# Autodesk Inventor assembly: FINAL ASSEMBLY CONNECTORS IN
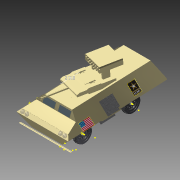
[picture p0: Inventor's stored thumbnail of the model, 180x180]
Saved by Autodesk Inventor 2015 (Build 190159000, 159)
## iProperties
Created: 2015-04-25
Part Number: FINAL ASSEMBLY CONNECTORS IN
Document SubType Name: Assembly
Designer: Simrun
Author: Simrun
## Documents named in this file (11)
- C:\Users\Simrun\Desktop\ALL M1117 Parts\FINAL ASSEMBLY CONNECTORS IN.iam
- C:\Users\Simrun\Desktop\ALL M1117 Parts\Correct middle piece Thursday 16.ipt
- C:\Users\Simrun\Desktop\ALL M1117 Parts\WORKING FRONT PART SPACESHIP COPY.ipt
- C:\Users\Simrun\Desktop\ALL M1117 Parts\T9 One Block Socket.ipt
- C:\Users\Simrun\Desktop\ALL M1117 Parts\T9 Two Block Socket.ipt
- C:\Users\Simrun\Desktop\ALL M1117 Parts\T9 Connector.ipt
- C:\Users\Simrun\Desktop\ALL M1117 Parts\Correct BACK PIECE.ipt
- C:\Users\Simrun\Desktop\ALL M1117 Parts\NewImprovedAxilforWheel.ipt
- C:\Users\Simrun\Desktop\ALL M1117 Parts\New Cannon M117 Guardian (1).ipt
- C:\Users\Simrun\Desktop\ALL M1117 Parts\AFinalWheel.ipt
- C:\Users\Simrun\Desktop\ALL M1117 Parts\Light.ipt
## Components (23 placed, 10 different names)
1. Correct middle piece Thursday 16:1 — Flush:1, Flush:2, Flush:3, Flush:8, Flush:9, Mate:4, Flush:10, Mate:7, Flush:12, Flush:13, Mate:9, Flush:15, Flush:16, Flush:17, Flush:18, Flush:19, Flush:20, Mate:10, Insert:1
2. WORKING FRONT PART SPACESHIP COPY:1 — Mate:1, Flush:4, Flush:5, Mate:3, Flush:8, Flush:9, Mate:4, Flush:10, Insert:3, Insert:6, Insert:11, Insert:12, Insert:13, Insert:14
3. T9 One Block Socket:1 — Flush:1, Flush:2, Flush:3
4. T9 Two Block Socket:1 — Mate:1, Flush:4, Flush:5, Mate:2, Flush:6
5. T9 Connector:1 — Mate:2, Flush:6, Flush:7
6. Correct BACK PIECE:1 — Mate:5, Mate:6, Flush:11, Flush:15, Flush:16, Flush:17, Flush:18, Flush:19, Flush:20, Mate:10, Insert:4, Insert:5
7. T9 Connector:2 — Mate:8, Flush:14, Mate:9
8. T9 One Block Socket:2 — Mate:5, Mate:6, Flush:11
9. T9 Two Block Socket:2 — Mate:7, Flush:12, Flush:13, Mate:8, Flush:14
10. NewImprovedAxilforWheel:1 — Insert:1, Insert:2
11. NewImprovedAxilforWheel:2 — Insert:5, Insert:7
12. NewImprovedAxilforWheel:3 — Insert:6, Insert:8
13. NewImprovedAxilforWheel:4 — Insert:4, Insert:9
14. NewImprovedAxilforWheel:5 — Insert:3, Insert:10
15. New Cannon M117 Guardian (1):1 — Insert:2
16. AFinalWheel:1 — Insert:8
17. AFinalWheel:2 — Insert:7
18. AFinalWheel:3 — Insert:9
19. AFinalWheel:4 — Insert:10
20. Light:1 — Insert:11
21. Light:2 — Insert:12
22. Light:3 — Insert:13
23. Light:4 — Insert:14
## Relationships (44: Flush 20, Insert 14, Mate 10)
- Flush:1: Correct middle piece Thursday 16:1 ↔ T9 One Block Socket:1
- Flush:2: Correct middle piece Thursday 16:1 ↔ T9 One Block Socket:1
- Flush:3: Correct middle piece Thursday 16:1 ↔ T9 One Block Socket:1
- Mate:1: WORKING FRONT PART SPACESHIP COPY:1 ↔ T9 Two Block Socket:1
- Flush:4: WORKING FRONT PART SPACESHIP COPY:1 ↔ T9 Two Block Socket:1
- Flush:5: WORKING FRONT PART SPACESHIP COPY:1 ↔ T9 Two Block Socket:1
- Mate:2: T9 Two Block Socket:1 ↔ T9 Connector:1
- Flush:6: T9 Two Block Socket:1 ↔ T9 Connector:1
- Flush:7: T9 Connector:1
- Mate:3: WORKING FRONT PART SPACESHIP COPY:1
- Flush:8: Correct middle piece Thursday 16:1 ↔ WORKING FRONT PART SPACESHIP COPY:1
- Flush:9: Correct middle piece Thursday 16:1 ↔ WORKING FRONT PART SPACESHIP COPY:1
- Mate:4: Correct middle piece Thursday 16:1 ↔ WORKING FRONT PART SPACESHIP COPY:1
- Flush:10: Correct middle piece Thursday 16:1 ↔ WORKING FRONT PART SPACESHIP COPY:1
- Mate:5: Correct BACK PIECE:1 ↔ T9 One Block Socket:2
- Mate:6: Correct BACK PIECE:1 ↔ T9 One Block Socket:2
- Flush:11: Correct BACK PIECE:1 ↔ T9 One Block Socket:2
- Mate:7: Correct middle piece Thursday 16:1 ↔ T9 Two Block Socket:2
- Flush:12: Correct middle piece Thursday 16:1 ↔ T9 Two Block Socket:2
- Flush:13: Correct middle piece Thursday 16:1 ↔ T9 Two Block Socket:2
- Mate:8: T9 Connector:2 ↔ T9 Two Block Socket:2
- Flush:14: T9 Connector:2 ↔ T9 Two Block Socket:2
- Mate:9: Correct middle piece Thursday 16:1 ↔ T9 Connector:2
- Flush:15: Correct middle piece Thursday 16:1 ↔ Correct BACK PIECE:1
- Flush:16: Correct middle piece Thursday 16:1 ↔ Correct BACK PIECE:1
- Flush:17: Correct middle piece Thursday 16:1 ↔ Correct BACK PIECE:1
- Flush:18: Correct middle piece Thursday 16:1 ↔ Correct BACK PIECE:1
- Flush:19: Correct middle piece Thursday 16:1 ↔ Correct BACK PIECE:1
- Flush:20: Correct middle piece Thursday 16:1 ↔ Correct BACK PIECE:1
- Mate:10: Correct middle piece Thursday 16:1 ↔ Correct BACK PIECE:1
- Insert:1: Correct middle piece Thursday 16:1 ↔ NewImprovedAxilforWheel:1
- Insert:2: NewImprovedAxilforWheel:1 ↔ New Cannon M117 Guardian (1):1
- Insert:3: WORKING FRONT PART SPACESHIP COPY:1 ↔ NewImprovedAxilforWheel:5
- Insert:4: Correct BACK PIECE:1 ↔ NewImprovedAxilforWheel:4
- Insert:5: Correct BACK PIECE:1 ↔ NewImprovedAxilforWheel:2
- Insert:6: WORKING FRONT PART SPACESHIP COPY:1 ↔ NewImprovedAxilforWheel:3
- Insert:7: NewImprovedAxilforWheel:2 ↔ AFinalWheel:2
- Insert:8: NewImprovedAxilforWheel:3 ↔ AFinalWheel:1
- Insert:9: NewImprovedAxilforWheel:4 ↔ AFinalWheel:3
- Insert:10: NewImprovedAxilforWheel:5 ↔ AFinalWheel:4
- Insert:11: WORKING FRONT PART SPACESHIP COPY:1 ↔ Light:1
- Insert:12: WORKING FRONT PART SPACESHIP COPY:1 ↔ Light:2
- Insert:13: WORKING FRONT PART SPACESHIP COPY:1 ↔ Light:3
- Insert:14: WORKING FRONT PART SPACESHIP COPY:1 ↔ Light:4
